# Autodesk Inventor assembly: Assembly2
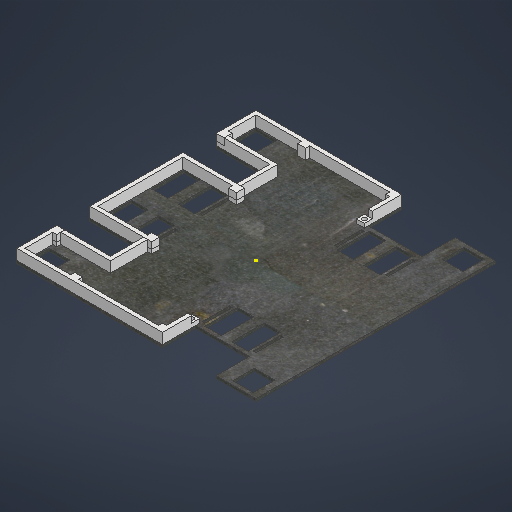
[picture p0: Inventor's stored thumbnail of the model, 512x512]
Saved by Autodesk Inventor 2026.2 (Build 302298010, 298A)
## iProperties
Created: 2026-09-07
Part Number: Assembly2
Document SubType Name: Assembly
Designer: karol
Author: karol
## Documents named in this file (7)
- C:\Users\karol\OneDrive\Dokumenty\GitHub\bolt_v2\ bolt_v2\CAD\Assemblys\mainassembly2.iam
- C:\Users\karol\OneDrive\Dokumenty\GitHub\bolt_v2\ bolt_v2\CAD\ready parts\base2.ipt
- C:\Users\karol\OneDrive\Dokumenty\GitHub\bolt_v2\ bolt_v2\CAD\ready parts\bmw2.ipt
- C:\Users\karol\OneDrive\Dokumenty\GitHub\bolt_v2\ bolt_v2\CAD\ready parts\left\leftbmw2.ipt
- C:\Users\karol\OneDrive\Dokumenty\GitHub\bolt_v2\ bolt_v2\CAD\ready parts\right\rightbmw.ipt
- C:\Users\karol\OneDrive\Dokumenty\GitHub\bolt_v2\ bolt_v2\CAD\ready parts\left\leftwall2.ipt
- C:\Users\karol\OneDrive\Dokumenty\GitHub\bolt_v2\ bolt_v2\CAD\ready parts\right\rightwall2.ipt
## Components (6 placed, 6 different names)
1. base2:1 — Flush:1, Flush:2, Flush:3, Flush:4, Flush:5, Flush:6, Flush:7
2. bmw2:1 — Flush:1
3. leftbmw2:1 — Flush:2, Flush:3
4. rightbmw:1 — Flush:4, Flush:5
5. leftwall2:1 — Flush:6
6. rightwall2:1 — Flush:7
## Relationships (7: Flush 7)
- Flush:1: base2:1 ↔ bmw2:1
- Flush:2: base2:1 ↔ leftbmw2:1
- Flush:3: base2:1 ↔ leftbmw2:1
- Flush:4: base2:1 ↔ rightbmw:1
- Flush:5: base2:1 ↔ rightbmw:1
- Flush:6: base2:1 ↔ leftwall2:1
- Flush:7: base2:1 ↔ rightwall2:1
